# Autodesk Inventor assembly: GuideDemo
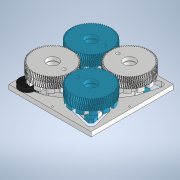
[picture p0: Inventor's stored thumbnail of the model, 180x180]
Saved by Autodesk Inventor 2020.2 (Build 242310000, 310)
## iProperties
Created: 2020-09-20
Part Number: GuideDemo
Document SubType Name: Assembly
Designer: elmar
Author: elmar
## Documents named in this file (7)
- D:\FourWireBraidingMachine\Documentation\GuideDemo.iam
- D:\FourWireBraidingMachine\InventorFiles\GuidePlateV1.ipt
- D:\FourWireBraidingMachine\InventorFiles\TipSpring.ipt
- D:\FourWireBraidingMachine\InventorFiles\HornGear.ipt
- D:\FourWireBraidingMachine\InventorFiles\HornGearMirror.ipt
- D:\FourWireBraidingMachine\InventorFiles\CarriagePlate.ipt
- D:\FourWireBraidingMachine\InventorFiles\SpoolHolder.ipt
## Components (17 placed, 6 different names)
1. GuidePlateV1:1 — Flush:1, Mate:1, Insert:1, Insert:2, Insert:3, Insert:4, Mate:2, Mate:3, Mate:4, Mate:5, Mate:6, Mate:7, Mate:8, Mate:9, Tangent:3, Tangent:4, Tangent:6, Tangent:7, Angle:3, Angle:4, Tangent:10, Tangent:11, Tangent:13, Tangent:14
2. HornGear:1 — Insert:3, Angle:2, Tangent:5, Tangent:12
3. HornGear:2 — Insert:4, Angle:2, Angle:4, Tangent:8, Tangent:9
4. HornGearMirror:1 — Insert:1, Angle:1, Angle:3
5. HornGearMirror:2 — Insert:2, Angle:1
6. CarriagePlate:1 — Mate:2, Insert:6
7. CarriagePlate:2 — Mate:3, Mate:4, Insert:7
8. CarriagePlate:3 — Insert:8, Mate:9
9. CarriagePlate:4 — Mate:5, Insert:5
10. SpoolHolder:1 — Insert:8, Tangent:3, Tangent:4, Tangent:5
11. SpoolHolder:2 — Insert:5, Tangent:12, Tangent:13, Tangent:14
12. SpoolHolder:3 — Insert:6, Tangent:6, Tangent:7, Tangent:8
13. SpoolHolder:4 — Insert:7, Tangent:9, Tangent:10, Tangent:11
14. TipSpring:1 — Flush:1, Mate:1
15. TipSpring:2
16. TipSpring:3
17. TipSpring:4
## Component patterns: (4 elements, first: TipSpring:1)
## Relationships (34: Tangent 12, Mate 9, Insert 8, Angle 4, Flush 1)
- Flush:1: GuidePlateV1:1 ↔ TipSpring:1
- Mate:1: GuidePlateV1:1 ↔ TipSpring:1
- Insert:1 (11 mm): GuidePlateV1:1 ↔ HornGearMirror:1
- Insert:2 (11 mm): GuidePlateV1:1 ↔ HornGearMirror:2
- Insert:3 (11 mm): GuidePlateV1:1 ↔ HornGear:1
- Insert:4 (11 mm): GuidePlateV1:1 ↔ HornGear:2
- Angle:1 (180 deg): HornGearMirror:1 ↔ HornGearMirror:2
- Angle:2 (180 deg): HornGear:1 ↔ HornGear:2
- Mate:2: GuidePlateV1:1 ↔ CarriagePlate:1
- Mate:3: GuidePlateV1:1 ↔ CarriagePlate:2
- Mate:4: GuidePlateV1:1 ↔ CarriagePlate:2
- Mate:5: GuidePlateV1:1 ↔ CarriagePlate:4
- Mate:6: GuidePlateV1:1
- Mate:7: GuidePlateV1:1
- Mate:8: GuidePlateV1:1
- Insert:5: CarriagePlate:4 ↔ SpoolHolder:2
- Insert:6: CarriagePlate:1 ↔ SpoolHolder:3
- Insert:7: CarriagePlate:2 ↔ SpoolHolder:4
- Insert:8: CarriagePlate:3 ↔ SpoolHolder:1
- Mate:9: GuidePlateV1:1 ↔ CarriagePlate:3
- Tangent:3: GuidePlateV1:1 ↔ SpoolHolder:1
- Tangent:4: GuidePlateV1:1 ↔ SpoolHolder:1
- Tangent:5: HornGear:1 ↔ SpoolHolder:1
- Tangent:6: GuidePlateV1:1 ↔ SpoolHolder:3
- Tangent:7: GuidePlateV1:1 ↔ SpoolHolder:3
- Angle:3 (5 deg): GuidePlateV1:1 ↔ HornGearMirror:1
- Angle:4 (5 deg): GuidePlateV1:1 ↔ HornGear:2
- Tangent:8: HornGear:2 ↔ SpoolHolder:3
- Tangent:9: HornGear:2 ↔ SpoolHolder:4
- Tangent:10: GuidePlateV1:1 ↔ SpoolHolder:4
- Tangent:11: GuidePlateV1:1 ↔ SpoolHolder:4
- Tangent:12: HornGear:1 ↔ SpoolHolder:2
- Tangent:13: GuidePlateV1:1 ↔ SpoolHolder:2
- Tangent:14: GuidePlateV1:1 ↔ SpoolHolder:2
